# Autodesk Inventor assembly: Лепестки со шпильками сборка
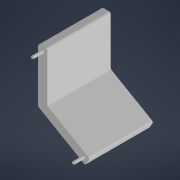
[picture p0: Inventor's stored thumbnail of the model, 180x180]
Saved by Autodesk Inventor 2022 (Build 260153000, 153)
## iProperties
Created: 2023-02-18
Part Number: Лепестки со шпильками сборка
Document SubType Name: Assembly
Designer: Глеб
Author: Глеб
## Documents named in this file (3)
- C:\Users\Глеб\Documents\Inventor\Файлы Inventor\Лепестки со шпильками сборка.iam
- C:\Users\Глеб\Documents\Inventor\Файлы Inventor\Шпилька для Лепестков.ipt
- C:\Users\Глеб\Documents\Inventor\Файлы Inventor\Лепесток БСП.ipt
## Components (3 placed, 2 different names)
1. Шпилька для Лепестков:1 — Совмещение:1, Совмещение:2
2. Лепесток БСП:1 — Совмещение:1, Совмещение:2, Совмещение:3, Совмещение:4
3. Шпилька для Лепестков:2 — Совмещение:3, Совмещение:4
## Relationships (4: Mate 4)
- Совмещение:1 [Mate]: Шпилька для Лепестков:1 ↔ Лепесток БСП:1
- Совмещение:2 [Mate] (12 mm): Шпилька для Лепестков:1 ↔ Лепесток БСП:1
- Совмещение:3 [Mate]: Лепесток БСП:1 ↔ Шпилька для Лепестков:2
- Совмещение:4 [Mate] (12 mm): Лепесток БСП:1 ↔ Шпилька для Лепестков:2
